# Autodesk Inventor assembly: TelescopeAssembly.ipt
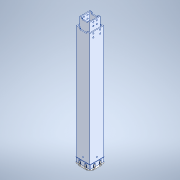
[picture p0: Inventor's stored thumbnail of the model, 180x180]
Saved by Autodesk Inventor 2022 (Build 260153000, 153)
## iProperties
Created: 2022-03-01
Part Number: TelescopeAssembly.ipt
Document SubType Name: Assembly
Designer: tagaz
Author: tagaz
## Documents named in this file (5)
- C:\Users\tagaz\OneDrive\Documents\T3-Cad\CAD\2022 Parts\TelescopeElev\TelescopeAssembly.ipt.iam
- C:\Users\tagaz\OneDrive\Documents\T3-Cad\CAD\2022 Parts\TelescopeElev\Telescoping elevator_p7.ipt
- C:\Users\tagaz\OneDrive\Documents\T3-Cad\CAD\2022 Parts\TelescopeElev\Telescoping elevator_stock3.ipt
- C:\Users\tagaz\OneDrive\Documents\T3-Cad\CAD\2022 Parts\TelescopeElev\Telescoping elevator_p5.ipt
- C:\Users\tagaz\OneDrive\Documents\T3-Cad\CAD\2022 Parts\TelescopeElev\Telescoping elevator_stock4.ipt
## Components (4 placed, 4 different names)
1. Telescoping elevator_p7:1 — Mate:5, Mate:6, Mate:7
2. Telescoping elevator_stock3:1 — Mate:5, Mate:6, Mate:7, Mate:16, Mate:17
3. Telescoping elevator_p5:1 — Mate:13, Mate:14, Mate:15
4. Telescoping elevator_stock4:1 — Mate:13, Mate:14, Mate:15, Mate:16, Mate:17
## Relationships (8: Mate 8)
- Mate:5: Telescoping elevator_p7:1 ↔ Telescoping elevator_stock3:1
- Mate:6: Telescoping elevator_p7:1 ↔ Telescoping elevator_stock3:1
- Mate:7: Telescoping elevator_p7:1 ↔ Telescoping elevator_stock3:1
- Mate:13: Telescoping elevator_p5:1 ↔ Telescoping elevator_stock4:1
- Mate:14: Telescoping elevator_p5:1 ↔ Telescoping elevator_stock4:1
- Mate:15: Telescoping elevator_p5:1 ↔ Telescoping elevator_stock4:1
- Mate:16 (3.175 mm): Telescoping elevator_stock3:1 ↔ Telescoping elevator_stock4:1
- Mate:17 (3.175 mm): Telescoping elevator_stock3:1 ↔ Telescoping elevator_stock4:1
